# Autodesk Inventor assembly: rotary encoder_chesr_2013
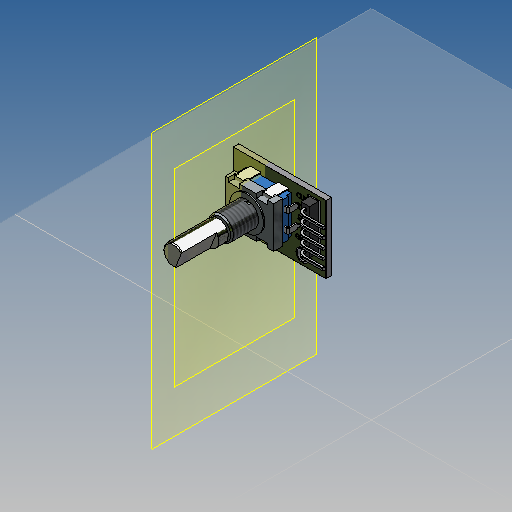
[picture p0: Inventor's stored thumbnail of the model, 512x512]
Saved by Autodesk Inventor 2019 (Build 230136000, 136)
## iProperties
Created: 2015-11-19
Part Number: rotary encoder_chesr_2013
Document SubType Name: Assembly
Designer: Tom
Mass: 2.35687 g
Surface Area: 43.4361 cm^2
Volume: 2.35687 cm^3
Density: 1 g/cm^3
Author: Tom
## Documents named in this file (11)
- C:\Users\User\Documents\Inventor\DayLightGlow\Rotary Encoder\rotary encoder_chesr_2013.iam
- C:\Users\User\Documents\Inventor\DayLightGlow\Rotary Encoder\pcb.ipt
- C:\Users\User\Documents\Inventor\DayLightGlow\Rotary Encoder\mtg flange.ipt
- C:\Users\User\Documents\Inventor\DayLightGlow\Rotary Encoder\body_encoder.ipt
- C:\Users\User\Documents\Inventor\DayLightGlow\Rotary Encoder\pins_encoder body_2.ipt
- C:\Users\User\Documents\Inventor\DayLightGlow\Rotary Encoder\5 pin header.ipt
- C:\Users\User\Documents\Inventor\DayLightGlow\Rotary Encoder\90d pin_header.ipt
- C:\Users\User\Documents\Inventor\DayLightGlow\Rotary Encoder\decal_encoder.ipt
- C:\Users\User\Documents\Inventor\DayLightGlow\Rotary Encoder\body_2.ipt
- C:\Users\User\Documents\Inventor\DayLightGlow\Rotary Encoder\shaft_encoder.ipt
- C:\Users\User\Documents\Inventor\DayLightGlow\Rotary Encoder\pins_encoder body_2_2.ipt
## Components (22 placed, 10 different names)
1. pcb:1 — Mate:1, Flush:2, Flush:3, Rotational:2, Mate:3, Rotational:3, Mate:4
2. mtg flange:1 — Rigid:1, Mate:5, Mate:7, Mate:9, Mate:10, Mate:12, Mate:13, Mate:15, Rotational:4, Flush:20
3. body_encoder:1 — Rigid:1, Mate:1, Flush:2, Flush:3, Mate:6, Mate:8, Mate:11, Mate:14, Mate:17, Flush:21, Mate:18, Mate:19
4. 5 pin header:1 — Rotational:2, Mate:3, Angle:1, Flush:12, Flush:13, Flush:14
5. decal_encoder:1 — Rotational:3, Mate:4
6. body_2:1 — Mate:5, Mate:6, Mate:7
7. body_2:2 — Mate:8, Mate:9, Mate:10
8. body_2:3 — Mate:11, Mate:12, Mate:13, Flush:15
9. body_2:4 — Mate:14, Flush:15, Mate:15
10. pins_encoder body_2:1 — Flush:17, Flush:18, Mate:17, Flush:20, Flush:21, Flush:22, Flush:23, Flush:24
11. pins_encoder body_2:2 — Flush:17, Flush:18, Flush:22
12. shaft_encoder:1 — Rotational:4
13. pins_encoder body_2_2:1
14. pins_encoder body_2_2:2
15. pins_encoder body_2:6 — Mate:18, Flush:23, Flush:24, Flush:25, Flush:26, Flush:27, Flush:28, Flush:29
16. pins_encoder body_2:7 — Flush:25, Flush:26, Mate:19
17. pins_encoder body_2:8 — Flush:27, Flush:28, Flush:29
18. 90d pin_header:1 — Angle:1, Flush:12, Flush:13, Flush:14
19. 90d pin_header:2
20. 90d pin_header:3
21. 90d pin_header:4
22. 90d pin_header:5
## Component patterns: (5 elements, first: 90d pin_header:1)
## Relationships (42: Flush 20, Mate 17, RevoluteJoint 3, WeldJoint 1, Angle 1)
- Rigid:1 [WeldJoint]: mtg flange:1 ↔ body_encoder:1
- Mate:1 (0.762 mm): pcb:1 ↔ body_encoder:1
- Flush:2 (4.572 mm): pcb:1 ↔ body_encoder:1
- Flush:3 (2.286 mm): pcb:1 ↔ body_encoder:1
- Rotational:2 [RevoluteJoint]: pcb:1 ↔ 5 pin header:1
- Mate:3: pcb:1 ↔ 5 pin header:1
- Angle:1 (0 deg): 5 pin header:1 ↔ 90d pin_header:1
- Flush:12 (-6.0452 mm): 5 pin header:1 ↔ 90d pin_header:1
- Flush:13 (0.889 mm): 5 pin header:1 ↔ 90d pin_header:1
- Flush:14 (-2.286 mm): 5 pin header:1 ↔ 90d pin_header:1
- Rotational:3 [RevoluteJoint]: pcb:1 ↔ decal_encoder:1
- Mate:4: pcb:1 ↔ decal_encoder:1
- Mate:5: mtg flange:1 ↔ body_2:1
- Mate:6: body_encoder:1 ↔ body_2:1
- Mate:7 (0.0635 mm): mtg flange:1 ↔ body_2:1
- Mate:8: body_encoder:1 ↔ body_2:2
- Mate:9: mtg flange:1 ↔ body_2:2
- Mate:10 (0.0635 mm): mtg flange:1 ↔ body_2:2
- Mate:11: body_encoder:1 ↔ body_2:3
- Mate:12: mtg flange:1 ↔ body_2:3
- Mate:13 (0.0635 mm): mtg flange:1 ↔ body_2:3
- Mate:14: body_encoder:1 ↔ body_2:4
- Flush:15: body_2:3 ↔ body_2:4
- Mate:15: mtg flange:1 ↔ body_2:4
- Flush:16 (-24.0284 mm)
- Flush:17: pins_encoder body_2:1 ↔ pins_encoder body_2:2
- Flush:18: pins_encoder body_2:1 ↔ pins_encoder body_2:2
- Rotational:4 [RevoluteJoint]: mtg flange:1 ↔ shaft_encoder:1
- Flush:19 (-24.0284 mm)
- Mate:17 (-0.635 mm): body_encoder:1 ↔ pins_encoder body_2:1
- Flush:20 (3.302 mm): mtg flange:1 ↔ pins_encoder body_2:1
- Flush:21 (2.3368 mm): body_encoder:1 ↔ pins_encoder body_2:1
- Flush:22 (5.08 mm): pins_encoder body_2:1 ↔ pins_encoder body_2:2
- Mate:18: body_encoder:1 ↔ pins_encoder body_2:6
- Flush:23: pins_encoder body_2:1 ↔ pins_encoder body_2:6
- Flush:24: pins_encoder body_2:1 ↔ pins_encoder body_2:6
- Flush:25: pins_encoder body_2:6 ↔ pins_encoder body_2:7
- Flush:26 (-5.08 mm): pins_encoder body_2:6 ↔ pins_encoder body_2:7
- Mate:19: body_encoder:1 ↔ pins_encoder body_2:7
- Flush:27: pins_encoder body_2:6 ↔ pins_encoder body_2:8
- Flush:28 (2.54 mm): pins_encoder body_2:6 ↔ pins_encoder body_2:8
- Flush:29: pins_encoder body_2:6 ↔ pins_encoder body_2:8
